# Autodesk Inventor assembly: Module
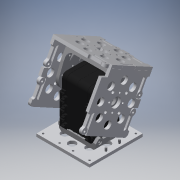
[picture p0: Inventor's stored thumbnail of the model, 180x180]
Saved by Autodesk Inventor 2016 (Build 200138000, 138)
## iProperties
Created: 2010-02-01
Part Number: Module
Document SubType Name: Assembly
Designer: Andrew
Translation Standard: STEP AP203
File Name: AX12_Fixed.STEP
Preprocessor: SolidWorks 2010
Postprocessor: Build: 254, Release: 2008 - Date: Fri 03/23/2007
Sent Units: MILLIMETERS
Uncertainty: 1e-05
Author: Andrew
## Documents named in this file (11)
- C:\Users\Rodrigo\Documents\2015-I\Tesis\Module\Module.iam
- C:\Users\Rodrigo\Documents\2015-I\Tesis\Dynamixel\AX12\AX12\ax12_wheel.ipt
- C:\Users\Rodrigo\Documents\2015-I\Tesis\Dynamixel\AX12\AX12\ax12_box.ipt
- C:\Users\Rodrigo\Documents\2015-I\Tesis\Dynamixel\AX12\AX12\ax12_cog.ipt
- C:\Users\Rodrigo\Documents\2015-I\Tesis\Dynamixel\F2\F2.ipt
- C:\Users\Rodrigo\Documents\2015-I\Tesis\Dynamixel\F3\F3.ipt
- C:\Users\Rodrigo\Documents\2015-I\Tesis\Module\Bottom.ipt
- C:\Users\Rodrigo\Documents\2015-I\Tesis\Module\Top.ipt
- C:\Users\Rodrigo\Documents\2015-I\Tesis\Module\Side.ipt
- C:\Users\Rodrigo\Documents\2015-I\Tesis\Module\SideB.ipt
- C:\Users\Rodrigo\Documents\2015-I\Tesis\Module\ScrewDummy.ipt
## Components (13 placed, 10 different names)
1. ax12_wheel:1 — Insert:1, Mate:1, Mate:2, Mate:3
2. ax12_box:1 — Insert:1, Mate:4, Mate:5, Mate:12
3. ax12_cog:1
4. F2:1 — Mate:1, Mate:2, Mate:3, Mate:6, Mate:7, Mate:8, Mate:13, Mate:14, Mate:15, Mate:16, Mate:17, Mate:18
5. F3:1 — Mate:4, Mate:5, Mate:9, Mate:10, Mate:11, Mate:12
6. Bottom:1 — Mate:6, Mate:7, Mate:8
7. Top:1 — Mate:9, Mate:10, Mate:11, Mate:19, Flush:1, Mate:20, Flush:2, Mate:21, Flush:3, Mate:22, Flush:4
8. Side:1 — Mate:13, Mate:14, Mate:15
9. SideB:1 — Mate:16, Mate:17, Mate:18
10. ScrewDummy:1 — Mate:19, Flush:1
11. ScrewDummy:2 — Mate:20, Flush:2
12. ScrewDummy:3 — Mate:21, Flush:3
13. ScrewDummy:4 — Mate:22, Flush:4
## Relationships (27: Mate 22, Flush 4, Insert 1)
- Insert:1: ax12_wheel:1 ↔ ax12_box:1
- Mate:1: ax12_wheel:1 ↔ F2:1
- Mate:2: ax12_wheel:1 ↔ F2:1
- Mate:3: ax12_wheel:1 ↔ F2:1
- Mate:4: ax12_box:1 ↔ F3:1
- Mate:5: ax12_box:1 ↔ F3:1
- Mate:6: F2:1 ↔ Bottom:1
- Mate:7: F2:1 ↔ Bottom:1
- Mate:8: F2:1 ↔ Bottom:1
- Mate:9: F3:1 ↔ Top:1
- Mate:10: F3:1 ↔ Top:1
- Mate:11: F3:1 ↔ Top:1
- Mate:12: ax12_box:1 ↔ F3:1
- Mate:13 (0.5 mm): F2:1 ↔ Side:1
- Mate:14: F2:1 ↔ Side:1
- Mate:15: F2:1 ↔ Side:1
- Mate:16 (0.5 mm): F2:1 ↔ SideB:1
- Mate:17: F2:1 ↔ SideB:1
- Mate:18: F2:1 ↔ SideB:1
- Mate:19: Top:1 ↔ ScrewDummy:1
- Flush:1: Top:1 ↔ ScrewDummy:1
- Mate:20: Top:1 ↔ ScrewDummy:2
- Flush:2: Top:1 ↔ ScrewDummy:2
- Mate:21: Top:1 ↔ ScrewDummy:3
- Flush:3: Top:1 ↔ ScrewDummy:3
- Mate:22: Top:1 ↔ ScrewDummy:4
- Flush:4: Top:1 ↔ ScrewDummy:4
